# Autodesk Inventor assembly: Extruder Assembly
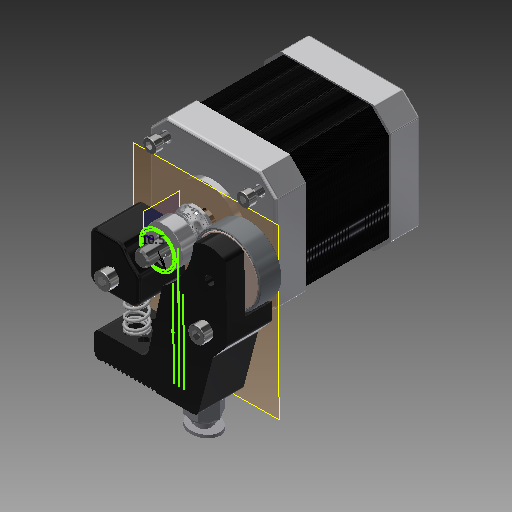
[picture p0: Inventor's stored thumbnail of the model, 512x512]
Saved by Autodesk Inventor 2018 (Build 220112000, 112)
## iProperties
Created: 2016-06-25
Part Number: Extruder Assembly
Document SubType Name: Assembly
Designer: joshmamo
Author: joshmamo
## Documents named in this file (11)
- C:\Users\Dan\OneDrive\SL-Inventor\The Beast v1.2 PackandGo\Workspaces\Workspace\Extruder Assembly.iam
- C:\Users\Dan\OneDrive\SL-Inventor\The Beast v1.2 PackandGo\Workspaces\Workspace\Spring Block.ipt
- C:\Users\Dan\OneDrive\SL-Inventor\The Beast v1.2 PackandGo\Workspaces\Workspace\Extruder Arm.ipt
- C:\Users\Dan\OneDrive\SL-Inventor\The Beast v1.2 PackandGo\Workspaces\Workspace\M1173041- NEMA 17.ipt
- C:\Users\Dan\OneDrive\SL-Inventor\The Beast v1.2 PackandGo\Workspaces\Workspace\608RS.ipt
- C:\Users\Dan\OneDrive\SL-Inventor\The Beast v1.2 PackandGo\Workspaces\Workspace\MK7.ipt
- C:\Users\Dan\OneDrive\SL-Inventor\The Beast v1.2 PackandGo\Workspaces\Workspace\Extruder Assembly\Design Accelerator\Compress Spring2.iam
- C:\Users\Dan\OneDrive\SL-Inventor\The Beast v1.2 PackandGo\Workspaces\Workspace\Pushfit-Adapter.iam
- C:\Users\Dan\OneDrive\SL-Inventor\The Beast v1.2 PackandGo\Workspaces\Workspace\en-US\ANSI B18.3.1M(6)\ANSI B18.3.1M - M3x0.5 x 25(1).ipt
- C:\Users\Dan\OneDrive\SL-Inventor\The Beast v1.2 PackandGo\Workspaces\Workspace\en-US\ANSI B18.3.1M(6)\ANSI B18.3.1M - M2.5x0.45 x 10(1).ipt
- C:\Users\Dan\OneDrive\SL-Inventor\The Beast v1.2 PackandGo\Workspaces\Workspace\en-US\ANSI B18.3.1M(6)\ANSI B18.3.1M - M3x0.5 x 20(1).ipt
## Components (11 placed, 10 different names)
1. Spring Block:1 — Mate:29, Mate:33, Mate:34, Mate:37, Mate:38
2. Extruder Arm:1 — Mate:23, Mate:24, Mate:35, Mate:36, Insert:3
3. M1173041- NEMA 17:1 — Mate:29, Mate:32, Flush:1
4. 608RS:1 — Mate:23, Mate:24
5. MK7:1 — Mate:32, Flush:1
6. Compress Spring:1 [sub-assembly] — Mate:33, Mate:34
7. Pushfit-Adapter:1 [sub-assembly] — Mate:35, Mate:36
8. Forged Socket Head Cap Screw - Metric M2.5x0.45 x 10:2
9. Forged Socket Head Cap Screw - Metric M2.5x0.45 x 10:1
10. Forged Socket Head Cap Screw - Metric M3x0.5 x 20:1 — Mate:37, Mate:38
11. Forged Socket Head Cap Screw - Metric M3x0.5 x 25:2 — Insert:3
## Relationships (12: Mate 10, Flush 1, Insert 1)
- Mate:23: Extruder Arm:1 ↔ 608RS:1
- Mate:24: Extruder Arm:1 ↔ 608RS:1
- Mate:29: Spring Block:1 ↔ M1173041- NEMA 17:1
- Mate:32: M1173041- NEMA 17:1 ↔ MK7:1
- Flush:1 (7.8 mm): M1173041- NEMA 17:1 ↔ MK7:1
- Mate:33: Spring Block:1 ↔ Compress Spring:1
- Mate:34: Spring Block:1 ↔ Compress Spring:1
- Mate:35: Extruder Arm:1 ↔ Pushfit-Adapter:1
- Mate:36: Extruder Arm:1 ↔ Pushfit-Adapter:1
- Mate:37: Spring Block:1 ↔ Forged Socket Head Cap Screw - Metric M3x0.5 x 20:1
- Mate:38: Spring Block:1 ↔ Forged Socket Head Cap Screw - Metric M3x0.5 x 20:1
- Insert:3: Extruder Arm:1 ↔ Forged Socket Head Cap Screw - Metric M3x0.5 x 25:2
